# Autodesk Inventor assembly: Matrix_12-0040
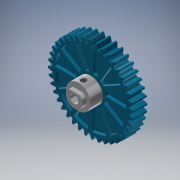
[picture p0: Inventor's stored thumbnail of the model, 180x180]
Saved by Autodesk Inventor 2017.1 (Build 211199000, 199)
## iProperties
Created: 2014-11-29
Part Number: Matrix_12-0040
Document SubType Name: Assembly
Designer: Philip
Author: Philip
## Documents named in this file (3)
- D:\FIRST\FTC KOP 2017\FTC 2017 KOP\Matrix\Matrix_12-0040.iam
- D:\FIRST\FTC KOP 2017\FTC 2017 KOP\Matrix\Matrix_12-0040_Gear.ipt
- D:\FIRST\FTC KOP 2017\FTC 2017 KOP\Matrix\Matrix_12-0040_Insert.ipt
## Components (2 placed, 2 different names)
1. Matrix_12-0040_Gear:1 — Insert:1
2. Matrix_12-0040_Insert:1 — Insert:1, Angle:1
## Relationships (2: Insert 1, Angle 1)
- Insert:1 (-0.5 mm): Matrix_12-0040_Gear:1 ↔ Matrix_12-0040_Insert:1
- Angle:1 (0 deg): Matrix_12-0040_Insert:1
